# Autodesk Inventor assembly: Full_Assembly
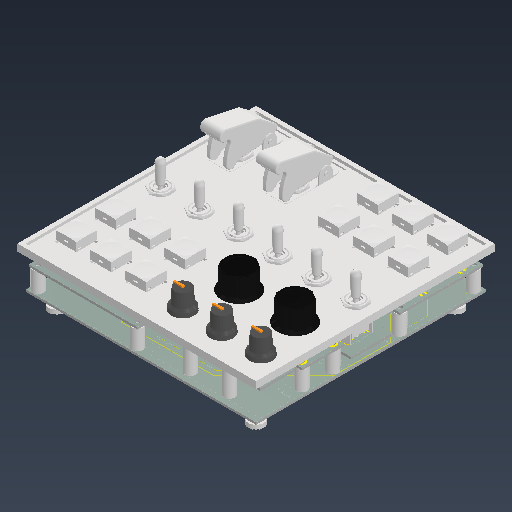
[picture p0: Inventor's stored thumbnail of the model, 512x512]
Saved by Autodesk Inventor 2025.3 (Build 293356000, 356)
## iProperties
Created: 2025-09-08
Part Number: Full_Assembly
Document SubType Name: Assembly
Designer: tolga
Author: tolga
## Documents named in this file (22)
- C:\Users\tolga\Documents\Repositories\Personal Projects\Sim-Control-Panel-v1.0\CAD\Full_Assembly.iam
- C:\Users\tolga\Documents\Repositories\Personal Projects\Sim-Control-Panel-v1.0\CAD\3rd_Party_Parts\On-On Switch.ipt
- C:\Users\tolga\Documents\Repositories\Personal Projects\Sim-Control-Panel-v1.0\CAD\3rd_Party_Parts\Switch Guard.ipt
- C:\Users\tolga\Documents\Repositories\Personal Projects\Sim-Control-Panel-v1.0\CAD\Faceplate.ipt
- C:\Users\tolga\Documents\Repositories\Personal Projects\Sim-Control-Panel-v1.0\CAD\3rd_Party_Parts\91862A525_Hex Panel Nut.ipt
- C:\Users\tolga\Documents\Repositories\Personal Projects\Sim-Control-Panel-v1.0\CAD\3rd_Party_Parts\Momentary Switch.ipt
- C:\Users\tolga\Documents\Repositories\Personal Projects\Sim-Control-Panel-v1.0\CAD\3rd_Party_Parts\PDB12-H4201-103BF\PDB12-H4201-103BF.iam
- C:\Users\tolga\Documents\Repositories\Personal Projects\Sim-Control-Panel-v1.0\CAD\3rd_Party_Parts\Potentiometer Knob.ipt
- C:\Users\tolga\Documents\Repositories\Personal Projects\Sim-Control-Panel-v1.0\CAD\3rd_Party_Parts\Encoder_Knob.ipt
- C:\Users\tolga\Documents\Repositories\Personal Projects\Sim-Control-Panel-v1.0\CAD\3rd_Party_Parts\PEC12R-4125F-N0012.ipt
- C:\Users\tolga\Documents\Repositories\Personal Projects\Sim-Control-Panel-v1.0\CAD\3rd_Party_Parts\Lighted_Buttons\Lighted_Buttons.iam
- C:\Users\tolga\Documents\Repositories\Personal Projects\Sim-Control-Panel-v1.0\CAD\3rd_Party_Parts\Bumpers.ipt
- C:\Users\tolga\Documents\Repositories\Personal Projects\Sim-Control-Panel-v1.0\CAD\Box.ipt
- C:\Users\tolga\Documents\Repositories\Personal Projects\Sim-Control-Panel-v1.0\CAD\Buttons_PCB\Buttons.iam
- C:\Users\tolga\Documents\Repositories\Personal Projects\Sim-Control-Panel-v1.0\CAD\Encoders_PCB\Encoders.iam
- C:\Users\tolga\Documents\Repositories\Personal Projects\Sim-Control-Panel-v1.0\CAD\Potentiometers_PCB\Potentiometers.iam
- C:\Users\tolga\Documents\Repositories\Personal Projects\Sim-Control-Panel-v1.0\CAD\Switches_PCB\Switches.iam
- C:\Users\tolga\Documents\Repositories\Personal Projects\Sim-Control-Panel-v1.0\CAD\Main_Panel_PCB\Main_Panel.iam
- C:\Users\tolga\Documents\Repositories\Personal Projects\Sim-Control-Panel-v1.0\CAD\Spacers\M3 4mm Generic Standoff.ipt
- C:\Users\tolga\Documents\Repositories\Personal Projects\Sim-Control-Panel-v1.0\CAD\Spacers\Button Spacer.ipt
- C:\Users\tolga\Documents\Repositories\Personal Projects\Sim-Control-Panel-v1.0\CAD\Spacers\Potentiometer Spacer.ipt
- C:\Users\tolga\Documents\Repositories\Personal Projects\Sim-Control-Panel-v1.0\CAD\Spacers\Encoder Spacer.ipt
## Components (82 placed, 21 different names)
1. Faceplate:1 — Insert:7, Angle:3, Insert:8, Angle:4, Insert:9, Insert:10, Insert:11, Angle:5, Insert:13, Insert:15, Insert:17, Insert:18, Mate:1, Mate:2, Flush:1, Mate:3, Mate:4, Flush:2, Mate:5, Mate:6, Flush:3
2. Switch Guard:2 — Insert:1, Angle:1, Insert:7, Angle:3
3. On-On Switch:4 — Insert:3, Angle:1
4. 91862A525_Hex Panel Nut:2 — Insert:1, Insert:3
5. Switch Guard:3 — Insert:8, Angle:4
6. On-On Switch:5
7. 91862A525_Hex Panel Nut:4
8. 91862A525_Hex Panel Nut:5 — Insert:9
9. 91862A525_Hex Panel Nut:6 — Insert:10
10. Box:1 — Mate:3, Mate:4, Flush:2, Insert:23, Insert:24, Insert:57, Insert:58, Insert:59, Insert:60
11. Encoders:1 [sub-assembly] — Mate:10, Insert:55, Insert:56
12. Potentiometers:1 [sub-assembly] — Mate:11, Insert:49, Insert:50
13. Switches:1 [sub-assembly] — Mate:12, Insert:25, Insert:26, Insert:27, Insert:28, Insert:29, Insert:30
14. Main_Panel:1 [sub-assembly] — Insert:23, Insert:24, Insert:31, Insert:32, Insert:37, Insert:38, Insert:43, Insert:44, Insert:45, Insert:46, Insert:47, Insert:48, Insert:51, Insert:52, Insert:53, Insert:54
15. M3 4mm Generic Standoff:6 — Insert:25, Insert:32
16. M3 4mm Generic Standoff:7 — Insert:26
17. M3 4mm Generic Standoff:8 — Insert:27
18. M3 4mm Generic Standoff:9 — Insert:28
19. M3 4mm Generic Standoff:10 — Insert:30, Insert:31
20. M3 4mm Generic Standoff:11 — Insert:29
21. Buttons:4 [sub-assembly] — Insert:33, Insert:34, Insert:35, Insert:36
22. Button Spacer:1 — Insert:36
23. Button Spacer:2 — Insert:35
24. Button Spacer:3 — Insert:33, Insert:37
25. Button Spacer:4 — Insert:34, Insert:38
26. Buttons:5 [sub-assembly]
27. Button Spacer:5 — Insert:44
28. Button Spacer:6
29. Button Spacer:7 — Insert:43
30. Button Spacer:8
31. Potentiometer Spacer:1 — Insert:45, Insert:49
32. Potentiometer Spacer:2 — Insert:46
33. Potentiometer Spacer:3 — Insert:47
34. Potentiometer Spacer:4 — Insert:48, Insert:50
35. Encoder Spacer:1 — Insert:51, Insert:56
36. Encoder Spacer:2 — Insert:52
37. Encoder Spacer:3 — Insert:53
38. Encoder Spacer:4 — Insert:54, Insert:55
39. Bumpers:1 — Insert:57
40. Bumpers:2 — Insert:59
41. Bumpers:3 — Insert:58
42. Bumpers:4 — Insert:60
43. Potentiometer Knob:1 — Insert:13, Insert:14
44. PDB12-H4201-103BF:1 [sub-assembly] — Insert:14, Mate:11
45. Potentiometer Knob:2
46. PDB12-H4201-103BF:2 [sub-assembly]
47. Potentiometer Knob:3
48. PDB12-H4201-103BF:3 [sub-assembly]
49. Encoder_Knob:1 — Insert:15, Insert:16
50. PEC12R-4125F-N0012:1 — Insert:16, Mate:10
51. Encoder_Knob:2
52. PEC12R-4125F-N0012:2
53. Momentary Switch:1 — Insert:11, Angle:5, Mate:12
54. 91862A525_Hex Panel Nut:8 — Insert:18
55. 91862A525_Hex Panel Nut:7 — Insert:17
56. Momentary Switch:2
57. 91862A525_Hex Panel Nut:9
58. 91862A525_Hex Panel Nut:10
59. Momentary Switch:3
60. 91862A525_Hex Panel Nut:11
61. 91862A525_Hex Panel Nut:12
62. Momentary Switch:4
63. 91862A525_Hex Panel Nut:13
64. 91862A525_Hex Panel Nut:14
65. Momentary Switch:5
66. 91862A525_Hex Panel Nut:15
67. 91862A525_Hex Panel Nut:16
68. Momentary Switch:6
69. 91862A525_Hex Panel Nut:17
70. 91862A525_Hex Panel Nut:18
71. Lighted_Buttons:1 [sub-assembly] — Mate:1, Mate:2, Flush:1
72. Lighted_Buttons:2 [sub-assembly]
73. Lighted_Buttons:3 [sub-assembly]
74. Lighted_Buttons:4 [sub-assembly]
75. Lighted_Buttons:5 [sub-assembly]
76. Lighted_Buttons:6 [sub-assembly]
77. Lighted_Buttons:7 [sub-assembly] — Mate:5, Mate:6, Flush:3
78. Lighted_Buttons:8 [sub-assembly]
79. Lighted_Buttons:9 [sub-assembly]
80. Lighted_Buttons:10 [sub-assembly]
81. Lighted_Buttons:11 [sub-assembly]
82. Lighted_Buttons:12 [sub-assembly]
## Component patterns: (3 elements, first: Potentiometer Knob:1 + PDB12-H4201-103BF:1), (2 elements, first: Encoder_Knob:1 + PEC12R-4125F-N0012:1), (6 elements, first: Momentary Switch:1 + 91862A525_Hex Panel Nut:8 + 91862A525_Hex Panel Nut:7), (6 elements, first: Lighted_Buttons:1), (6 elements, first: Lighted_Buttons:7)
## Relationships (70: Insert 53, Mate 9, Angle 5, Flush 3)
- Insert:1: Switch Guard:2 ↔ 91862A525_Hex Panel Nut:2
- Insert:3 (-0.3 mm): On-On Switch:4 ↔ 91862A525_Hex Panel Nut:2
- Angle:1 (-90 deg): Switch Guard:2 ↔ On-On Switch:4
- [Insert]: Switch Guard:3 ↔ 91862A525_Hex Panel Nut:4
- [Insert] (-0.3 mm): On-On Switch:5 ↔ 91862A525_Hex Panel Nut:4
- [Angle] (-90 deg): Switch Guard:3 ↔ On-On Switch:5
- Insert:7: Faceplate:1 ↔ Switch Guard:2
- Angle:3 (0 deg): Faceplate:1 ↔ Switch Guard:2
- Insert:8: Faceplate:1 ↔ Switch Guard:3
- Angle:4 (180 deg): Faceplate:1 ↔ Switch Guard:3
- Insert:9: Faceplate:1 ↔ 91862A525_Hex Panel Nut:5
- Insert:10: Faceplate:1 ↔ 91862A525_Hex Panel Nut:6
- Insert:11 (-2.18 mm): Faceplate:1 ↔ Momentary Switch:1
- Angle:5 (0 deg): Faceplate:1 ↔ Momentary Switch:1
- Insert:13 (1 mm): Faceplate:1 ↔ Potentiometer Knob:1
- Insert:14 (1.6 mm): Potentiometer Knob:1 ↔ PDB12-H4201-103BF:1
- Insert:15 (1 mm): Faceplate:1 ↔ Encoder_Knob:1
- Insert:16: Encoder_Knob:1 ↔ PEC12R-4125F-N0012:1
- Insert:17: Faceplate:1 ↔ 91862A525_Hex Panel Nut:7
- Insert:18: Faceplate:1 ↔ 91862A525_Hex Panel Nut:8
- Mate:1: Faceplate:1 ↔ Lighted_Buttons:1
- Mate:2: Faceplate:1 ↔ Lighted_Buttons:1
- Flush:1 (1 mm): Faceplate:1 ↔ Lighted_Buttons:1
- Mate:3 (0.1 mm): Faceplate:1 ↔ Box:1
- Mate:4 (0.1 mm): Faceplate:1 ↔ Box:1
- Flush:2: Faceplate:1 ↔ Box:1
- Mate:5: Faceplate:1 ↔ Lighted_Buttons:7
- Mate:6: Faceplate:1 ↔ Lighted_Buttons:7
- Flush:3 (1 mm): Faceplate:1 ↔ Lighted_Buttons:7
- Mate:10: Encoders:1 ↔ PEC12R-4125F-N0012:1
- Mate:11: Potentiometers:1 ↔ PDB12-H4201-103BF:1
- Mate:12: Switches:1 ↔ Momentary Switch:1
- Insert:23: Box:1 ↔ Main_Panel:1
- Insert:24: Box:1 ↔ Main_Panel:1
- Insert:25: Switches:1 ↔ M3 4mm Generic Standoff:6
- Insert:26: Switches:1 ↔ M3 4mm Generic Standoff:7
- Insert:27: Switches:1 ↔ M3 4mm Generic Standoff:8
- Insert:28: Switches:1 ↔ M3 4mm Generic Standoff:9
- Insert:29: Switches:1 ↔ M3 4mm Generic Standoff:11
- Insert:30: Switches:1 ↔ M3 4mm Generic Standoff:10
- Insert:31: Main_Panel:1 ↔ M3 4mm Generic Standoff:10
- Insert:32: Main_Panel:1 ↔ M3 4mm Generic Standoff:6
- Insert:33: Buttons:4 ↔ Button Spacer:3
- Insert:34: Buttons:4 ↔ Button Spacer:4
- Insert:35: Buttons:4 ↔ Button Spacer:2
- Insert:36: Buttons:4 ↔ Button Spacer:1
- Insert:37: Main_Panel:1 ↔ Button Spacer:3
- Insert:38: Main_Panel:1 ↔ Button Spacer:4
- [Insert]: Buttons:5 ↔ Button Spacer:7
- [Insert]: Buttons:5 ↔ Button Spacer:8
- [Insert]: Buttons:5 ↔ Button Spacer:6
- [Insert]: Buttons:5 ↔ Button Spacer:5
- Insert:43: Main_Panel:1 ↔ Button Spacer:7
- Insert:44: Main_Panel:1 ↔ Button Spacer:5
- Insert:45: Main_Panel:1 ↔ Potentiometer Spacer:1
- Insert:46: Main_Panel:1 ↔ Potentiometer Spacer:2
- Insert:47: Main_Panel:1 ↔ Potentiometer Spacer:3
- Insert:48: Main_Panel:1 ↔ Potentiometer Spacer:4
- Insert:49: Potentiometers:1 ↔ Potentiometer Spacer:1
- Insert:50: Potentiometers:1 ↔ Potentiometer Spacer:4
- Insert:51: Main_Panel:1 ↔ Encoder Spacer:1
- Insert:52: Main_Panel:1 ↔ Encoder Spacer:2
- Insert:53: Main_Panel:1 ↔ Encoder Spacer:3
- Insert:54: Main_Panel:1 ↔ Encoder Spacer:4
- Insert:55: Encoders:1 ↔ Encoder Spacer:4
- Insert:56: Encoders:1 ↔ Encoder Spacer:1
- Insert:57: Box:1 ↔ Bumpers:1
- Insert:58: Box:1 ↔ Bumpers:3
- Insert:59: Box:1 ↔ Bumpers:2
- Insert:60: Box:1 ↔ Bumpers:4
## Named parameters: d70_d66 = 0 mm, d72_d68 = -0.3 mm, d73_d69 = -90 deg, d157_d152 = 0 mm, d158_d153 = 0 mm, d159_d154 = 0 mm, d160_d151 = 0 mm
